# Autodesk Inventor assembly: enc-SidePanel Mitte - Assembly no Absorber
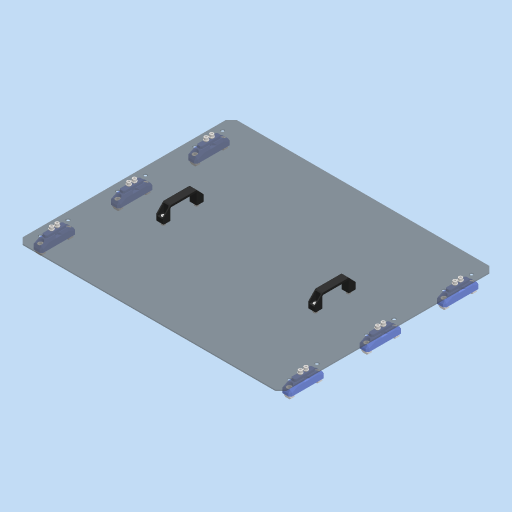
[picture p0: Inventor's stored thumbnail of the model, 512x512]
Saved by Autodesk Inventor 2023.2 (Build 272271000, 271)
## iProperties
Created: 2023-11-30
Part Number: enc-SidePanel Mitte - Assembly no Absorber
Document SubType Name: Assembly
Designer: Nils Bade
Author: Nils Bade
## Documents named in this file (6)
- C:\Users\nilsb\Documents\Inventor\Projektarbeit-Bade\Enclosure\enc-SidePanel Mitte - Assembly no Absorber.iam
- C:\Users\nilsb\Documents\Inventor\Projektarbeit-Bade\Enclosure\enc-SidePanel Mitte 500x708.ipt
- C:\Users\nilsb\Documents\Inventor\Projektarbeit-Bade\Enclosure\V-Slot Door Handle v1.ipt
- C:\Users\nilsb\Documents\Inventor\Projektarbeit-Bade\Enclosure\Magnet PanelFrame Straight connected.iam
- C:\Users\nilsb\Documents\Inventor\Projektarbeit-Bade\Schrauben\Cap Head Screw M6x16 - DIN912.ipt
- C:\Users\nilsb\Documents\Inventor\Projektarbeit-Bade\RatRig_Standards\Hex Locking Nut - M6 v2.ipt
## Components (17 placed, 5 different names)
1. enc-SidePanel Mitte 575x708:1 — Passend:1, Passend:2, Passend:3, Passend:4, Passend:5, Passend:6, Passend:7, Passend:8, Passend:9, Passend:10, Passend:11, Passend:12, Passend:13, Passend:14, Passend:15, Passend:16, Passend:17, Passend:18, Passend:19, Passend:20, Passend:21, Passend:22, Passend:23, Passend:24, Passend:37, Passend:38, Passend:39, Passend:40
2. V-Slot Door Handle v1:1 — Passend:1, Passend:2, Passend:5, Passend:25, Passend:26, Passend:29, Passend:30
3. V-Slot Door Handle v1:2 — Passend:3, Passend:4, Passend:6, Passend:27, Passend:28, Passend:31, Passend:32
4. Magnet PanelFrame Straight connected:1 [sub-assembly] — Passend:7, Passend:8, Passend:9
5. Magnet PanelFrame Straight connected:2 [sub-assembly] — Passend:10, Passend:11, Passend:12
6. Magnet PanelFrame Straight connected:3 [sub-assembly] — Passend:13, Passend:14, Passend:15
7. Magnet PanelFrame Straight connected:4 [sub-assembly] — Passend:16, Passend:17, Passend:18
8. Magnet PanelFrame Straight connected:5 [sub-assembly] — Passend:19, Passend:20, Passend:21
9. Magnet PanelFrame Straight connected:6 [sub-assembly] — Passend:22, Passend:23, Passend:24
10. Cap Head Screw M6x16 - DIN912:1 — Passend:25, Passend:29, Passend:35
11. Cap Head Screw M6x16 - DIN912:2 — Passend:26, Passend:30, Passend:36
12. Cap Head Screw M6x16 - DIN912:3 — Passend:27, Passend:31, Passend:34
13. Cap Head Screw M6x16 - DIN912:4 — Passend:28, Passend:32, Passend:33
14. Hex Locking Nut - M6 v2:1 — Passend:33, Passend:38
15. Hex Locking Nut - M6 v2:2 — Passend:34, Passend:37
16. Hex Locking Nut - M6 v2:3 — Passend:35, Passend:39
17. Hex Locking Nut - M6 v2:4 — Passend:36, Passend:40
## Relationships (40: Mate 40)
- Passend:1 [Mate]: enc-SidePanel Mitte 575x708:1 ↔ V-Slot Door Handle v1:1
- Passend:2 [Mate]: enc-SidePanel Mitte 575x708:1 ↔ V-Slot Door Handle v1:1
- Passend:3 [Mate]: enc-SidePanel Mitte 575x708:1 ↔ V-Slot Door Handle v1:2
- Passend:4 [Mate]: enc-SidePanel Mitte 575x708:1 ↔ V-Slot Door Handle v1:2
- Passend:5 [Mate]: enc-SidePanel Mitte 575x708:1 ↔ V-Slot Door Handle v1:1
- Passend:6 [Mate]: enc-SidePanel Mitte 575x708:1 ↔ V-Slot Door Handle v1:2
- Passend:7 [Mate]: enc-SidePanel Mitte 575x708:1 ↔ Magnet PanelFrame Straight connected:1
- Passend:8 [Mate]: enc-SidePanel Mitte 575x708:1 ↔ Magnet PanelFrame Straight connected:1
- Passend:9 [Mate]: enc-SidePanel Mitte 575x708:1 ↔ Magnet PanelFrame Straight connected:1
- Passend:10 [Mate]: enc-SidePanel Mitte 575x708:1 ↔ Magnet PanelFrame Straight connected:2
- Passend:11 [Mate]: enc-SidePanel Mitte 575x708:1 ↔ Magnet PanelFrame Straight connected:2
- Passend:12 [Mate]: enc-SidePanel Mitte 575x708:1 ↔ Magnet PanelFrame Straight connected:2
- Passend:13 [Mate]: enc-SidePanel Mitte 575x708:1 ↔ Magnet PanelFrame Straight connected:3
- Passend:14 [Mate]: enc-SidePanel Mitte 575x708:1 ↔ Magnet PanelFrame Straight connected:3
- Passend:15 [Mate]: enc-SidePanel Mitte 575x708:1 ↔ Magnet PanelFrame Straight connected:3
- Passend:16 [Mate]: enc-SidePanel Mitte 575x708:1 ↔ Magnet PanelFrame Straight connected:4
- Passend:17 [Mate]: enc-SidePanel Mitte 575x708:1 ↔ Magnet PanelFrame Straight connected:4
- Passend:18 [Mate]: enc-SidePanel Mitte 575x708:1 ↔ Magnet PanelFrame Straight connected:4
- Passend:19 [Mate]: enc-SidePanel Mitte 575x708:1 ↔ Magnet PanelFrame Straight connected:5
- Passend:20 [Mate]: enc-SidePanel Mitte 575x708:1 ↔ Magnet PanelFrame Straight connected:5
- Passend:21 [Mate]: enc-SidePanel Mitte 575x708:1 ↔ Magnet PanelFrame Straight connected:5
- Passend:22 [Mate]: enc-SidePanel Mitte 575x708:1 ↔ Magnet PanelFrame Straight connected:6
- Passend:23 [Mate]: enc-SidePanel Mitte 575x708:1 ↔ Magnet PanelFrame Straight connected:6
- Passend:24 [Mate]: enc-SidePanel Mitte 575x708:1 ↔ Magnet PanelFrame Straight connected:6
- Passend:25 [Mate]: V-Slot Door Handle v1:1 ↔ Cap Head Screw M6x16 - DIN912:1
- Passend:26 [Mate]: V-Slot Door Handle v1:1 ↔ Cap Head Screw M6x16 - DIN912:2
- Passend:27 [Mate]: V-Slot Door Handle v1:2 ↔ Cap Head Screw M6x16 - DIN912:3
- Passend:28 [Mate]: V-Slot Door Handle v1:2 ↔ Cap Head Screw M6x16 - DIN912:4
- Passend:29 [Mate]: V-Slot Door Handle v1:1 ↔ Cap Head Screw M6x16 - DIN912:1
- Passend:30 [Mate]: V-Slot Door Handle v1:1 ↔ Cap Head Screw M6x16 - DIN912:2
- Passend:31 [Mate]: V-Slot Door Handle v1:2 ↔ Cap Head Screw M6x16 - DIN912:3
- Passend:32 [Mate]: V-Slot Door Handle v1:2 ↔ Cap Head Screw M6x16 - DIN912:4
- Passend:33 [Mate]: Cap Head Screw M6x16 - DIN912:4 ↔ Hex Locking Nut - M6 v2:1
- Passend:34 [Mate]: Cap Head Screw M6x16 - DIN912:3 ↔ Hex Locking Nut - M6 v2:2
- Passend:35 [Mate]: Cap Head Screw M6x16 - DIN912:1 ↔ Hex Locking Nut - M6 v2:3
- Passend:36 [Mate]: Cap Head Screw M6x16 - DIN912:2 ↔ Hex Locking Nut - M6 v2:4
- Passend:37 [Mate]: enc-SidePanel Mitte 575x708:1 ↔ Hex Locking Nut - M6 v2:2
- Passend:38 [Mate]: enc-SidePanel Mitte 575x708:1 ↔ Hex Locking Nut - M6 v2:1
- Passend:39 [Mate]: enc-SidePanel Mitte 575x708:1 ↔ Hex Locking Nut - M6 v2:3
- Passend:40 [Mate]: enc-SidePanel Mitte 575x708:1 ↔ Hex Locking Nut - M6 v2:4
